# Autodesk Inventor assembly: solar cleaning systam assly new
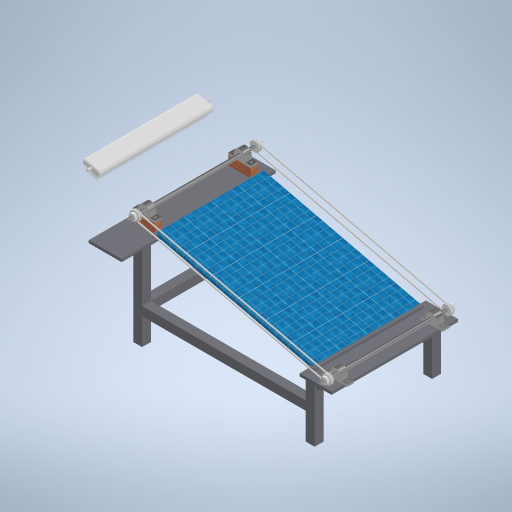
[picture p0: Inventor's stored thumbnail of the model, 512x512]
Saved by Autodesk Inventor 2024 (Build 280153000, 153)
## iProperties
Created: 2023-06-12
Part Number: solar cleaning systam assly new
Description: STEP AP203
Document SubType Name: Assembly
Designer: VICTUS
Sending System: SolidWorks 2019
Preprocessor: SwSTEP 2.0
Title: solar cleaning systam assly 2.STEP
Revision Number: ANY
## Documents named in this file (13)
- D:\WOE\Combined data\solar cleaning systam assly new.iam
- D:\WOE\Combined data\600x900 solar.ipt
- D:\WOE\Combined data\bearing block.ipt
- D:\WOE\Combined data\shaft 17x700.ipt
- D:\WOE\Combined data\pulley.ipt
- D:\WOE\Combined data\pulley - Copy.ipt
- D:\WOE\Combined data\WOODEN_Default_As Machined_.ipt
- D:\WOE\Combined data\WOODEN BLOCK.ipt
- D:\ADDUZ\STUDIES\WorldOfEngineering\Brush2.ipt
- D:\ADDUZ\STUDIES\WorldOfEngineering\motor_base.ipt
- D:\ADDUZ\STUDIES\WorldOfEngineering\f-130-motor-1.snapshot.1\scaledmotor.ipt
- D:\ADDUZ\STUDIES\WorldOfEngineering\drip pipe.ipt
- C:\Users\ASUS\OneDrive\Documents\Brush.ipt
## Components (19 placed, 19 different names)
1. 600x900 solar_1
2. bearing block_2 — Mate:3, Mate:4, Mate:5, Flush:1, Flush:2
3. bearing block_3 — Mate:2, Mate:6, Flush:3, Flush:4, Mate:7
4. shaft 17x700_4 — Mate:1, Mate:2, Mate:3, Mate:4, Mate:7, Mate:8, Mate:9, Mate:10, Mate:27
5. pulley_5 — Mate:1, Mate:8, Mate:22, Mate:24, Transitional:2
6. bearing block_6 — Mate:12, Mate:14, Mate:21, Flush:7
7. bearing block_7 — Mate:13, Mate:18, Mate:20
8. shaft 17x700_8 — Mate:12, Mate:13, Mate:14, Mate:15, Mate:16, Mate:17, Mate:18, Mate:19, Mate:23
9. pulley - Copy_9 — Mate:16, Mate:17
10. pulley_10 — Mate:9, Mate:10, Mate:23, Mate:25, Transitional:1
11. pulley - Copy_11 — Mate:15, Mate:19, Mate:22
12. WOODEN_Default<As Machined>_12 — Mate:11, Flush:5, Flush:6, Mate:20, Mate:21, Flush:7, Mate:26, Flush:8, Flush:9
13. WOODEN BLOCK_13 — Mate:5, Flush:1, Flush:2, Mate:11, Flush:5, Flush:6, Mate:29
14. WOODEN BLOCK_14 — Mate:6, Flush:3, Flush:4
15. Brush2:1 — Mate:24, Mate:25
16. motor_base:1 — Mate:26, Flush:8, Flush:9, Mate:28
17. scaledmotor:1 — Mate:27, Mate:28
18. drip pipe:1 — Mate:29
19. Brush:1 — Transitional:1, Transitional:2
## Relationships (40: Mate 29, Flush 9, Transitional 2)
- Mate:1: shaft 17x700_4 ↔ pulley_5
- Mate:2: bearing block_3 ↔ shaft 17x700_4
- Mate:3: bearing block_2 ↔ shaft 17x700_4
- Mate:4: bearing block_2 ↔ shaft 17x700_4
- Mate:5: bearing block_2 ↔ WOODEN BLOCK_13
- Flush:1: bearing block_2 ↔ WOODEN BLOCK_13
- Flush:2: bearing block_2 ↔ WOODEN BLOCK_13
- Mate:6: bearing block_3 ↔ WOODEN BLOCK_14
- Flush:3: bearing block_3 ↔ WOODEN BLOCK_14
- Flush:4: bearing block_3 ↔ WOODEN BLOCK_14
- Mate:7: bearing block_3 ↔ shaft 17x700_4
- Mate:8: shaft 17x700_4 ↔ pulley_5
- Mate:9: shaft 17x700_4 ↔ pulley_10
- Mate:10: shaft 17x700_4 ↔ pulley_10
- Mate:11: WOODEN_Default<As Machined>_12 ↔ WOODEN BLOCK_13
- Flush:5 (29 mm): WOODEN_Default<As Machined>_12 ↔ WOODEN BLOCK_13
- Flush:6 (-67 mm): WOODEN_Default<As Machined>_12 ↔ WOODEN BLOCK_13
- Mate:12: bearing block_6 ↔ shaft 17x700_8
- Mate:13: bearing block_7 ↔ shaft 17x700_8
- Mate:14: bearing block_6 ↔ shaft 17x700_8
- Mate:15: shaft 17x700_8 ↔ pulley - Copy_11
- Mate:16: shaft 17x700_8 ↔ pulley - Copy_9
- Mate:17: shaft 17x700_8 ↔ pulley - Copy_9
- Mate:18: bearing block_7 ↔ shaft 17x700_8
- Mate:19: shaft 17x700_8 ↔ pulley - Copy_11
- Mate:20: bearing block_7 ↔ WOODEN_Default<As Machined>_12
- Mate:21: bearing block_6 ↔ WOODEN_Default<As Machined>_12
- Mate:22: pulley_5 ↔ pulley - Copy_11
- Mate:23: shaft 17x700_8 ↔ pulley_10
- Flush:7 (67 mm): bearing block_6 ↔ WOODEN_Default<As Machined>_12
- Mate:24: pulley_5 ↔ Brush2:1
- Mate:25: pulley_10 ↔ Brush2:1
- Mate:26: WOODEN_Default<As Machined>_12 ↔ motor_base:1
- Flush:8: WOODEN_Default<As Machined>_12 ↔ motor_base:1
- Flush:9: WOODEN_Default<As Machined>_12 ↔ motor_base:1
- Mate:27: shaft 17x700_4 ↔ scaledmotor:1
- Mate:28: motor_base:1 ↔ scaledmotor:1
- Mate:29: WOODEN BLOCK_13 ↔ drip pipe:1
- Transitional:1: pulley_10 ↔ Brush:1
- Transitional:2: pulley_5 ↔ Brush:1
